# Autodesk Inventor assembly: 3xCombiner
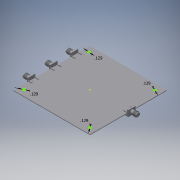
[picture p0: Inventor's stored thumbnail of the model, 180x180]
Saved by Autodesk Inventor 2018 (Build 220112000, 112)
## iProperties
Created: 2018-04-06
Part Number: 3xCombiner
Document SubType Name: Assembly
Designer: bbramman
Author: bbramman
## Documents named in this file (3)
- C:\Users\bbramman\OneDrive\Documents\Trapped Ion Research (Grad)\Electronics\pll-evalboard-synthesizer\Box CAD\3xCombiner.iam
- C:\Users\bbramman\OneDrive\Documents\Trapped Ion Research (Grad)\Electronics\pll-evalboard-synthesizer\Box CAD\3xCombiner.ipt
- C:\Users\bbramman\OneDrive\Documents\Trapped Ion Research (Grad)\Electronics\pll-evalboard-synthesizer\Box CAD\SMA-END.ipt
## Components (5 placed, 2 different names)
1. 3xCombiner:1 — Mate:1, Mate:2, Flush:1, Mate:3, Mate:4, Mate:5, Flush:2, Mate:6, Mate:7, Mate:8
2. SMA-END:1 — Mate:5, Mate:8
3. SMA-END:2 — Mate:4, Flush:2, Mate:6
4. SMA-END:3 — Mate:3, Mate:7
5. SMA-END:4 — Mate:1, Mate:2, Flush:1
## Relationships (10: Mate 8, Flush 2)
- Mate:1: 3xCombiner:1 ↔ SMA-END:4
- Mate:2: 3xCombiner:1 ↔ SMA-END:4
- Flush:1 (48.26 mm): 3xCombiner:1 ↔ SMA-END:4
- Mate:3: 3xCombiner:1 ↔ SMA-END:3
- Mate:4: 3xCombiner:1 ↔ SMA-END:2
- Mate:5: 3xCombiner:1 ↔ SMA-END:1
- Flush:2 (48.26 mm): 3xCombiner:1 ↔ SMA-END:2
- Mate:6: 3xCombiner:1 ↔ SMA-END:2
- Mate:7: 3xCombiner:1 ↔ SMA-END:3
- Mate:8: 3xCombiner:1 ↔ SMA-END:1
